# Autodesk Inventor assembly: liftMotorWithPotMounted
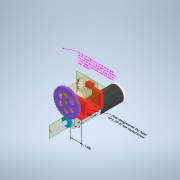
[picture p0: Inventor's stored thumbnail of the model, 180x180]
Saved by Autodesk Inventor 2020.2 (Build 242310000, 310)
## iProperties
Created: 2019-11-21
Part Number: liftMotorWithPotMounted
Document SubType Name: Assembly
Designer: steele
Author: steele
## Documents named in this file (9)
- C:\git\CAD-Development\robSteele\liftSpool\liftMotorWithPotMounted.iam
- C:\git\CAD-Development\robSteele\liftSpool\am-3762 - 36_1 - CIM Sport.iam
- C:\git\CAD-Development\robSteele\liftSpool\plateForPot.ipt
- C:\git\CAD-Development\robSteele\liftSpool\PotHolderAssembly.iam
- C:\git\CAD-Development\robSteele\liftSpool\liftMotorWithPotMounted\Design Accelerator\Spur Gears1.iam
- C:\git\CAD-Development\robSteele\liftSpool\spoolV09.ipt
- C:\git\CAD-Development\robSteele\liftSpool\am-0255+2.5inch+CIM+Motor.ipt
- C:\git\CAD-Development\robSteele\liftSpool\WormGearDriveForPot.iam
- C:\git\CAD-Development\robSteele\liftSpool\3_8_inchSteelShaft.ipt
## Components (8 placed, 8 different names)
1. am-3762 - 36_1 - CIM Sport:1 [sub-assembly] — Mate:1, Mate:2, Mate:3, Insert:1, Flush:1, Insert:2, Mate:4, Mate:5
2. plateForPot:1 — Mate:1, Mate:2, Mate:3
3. PotHolderAssembly:1 [sub-assembly] — Insert:5
4. Spur Gears:1 [sub-assembly] — Flush:1, Mate:4, Mate:5, Insert:3
5. spoolV09:1 — Insert:1
6. am-0255+2.5inch+CIM+Motor:1 — Insert:2
7. WormGearDriveForPot:1 [sub-assembly] — Insert:4, Insert:5
8. 3_8_inchSteelShaft:1 — Insert:3, Insert:4
## Relationships (11: Mate 5, Insert 5, Flush 1)
- Mate:1: am-3762 - 36_1 - CIM Sport:1 ↔ plateForPot:1
- Mate:2: am-3762 - 36_1 - CIM Sport:1 ↔ plateForPot:1
- Mate:3: am-3762 - 36_1 - CIM Sport:1 ↔ plateForPot:1
- Insert:1: am-3762 - 36_1 - CIM Sport:1 ↔ spoolV09:1
- Flush:1: am-3762 - 36_1 - CIM Sport:1 ↔ Spur Gears:1
- Insert:2: am-3762 - 36_1 - CIM Sport:1 ↔ am-0255+2.5inch+CIM+Motor:1
- Mate:4: am-3762 - 36_1 - CIM Sport:1 ↔ Spur Gears:1
- Mate:5: am-3762 - 36_1 - CIM Sport:1 ↔ Spur Gears:1
- Insert:3: Spur Gears:1 ↔ 3_8_inchSteelShaft:1
- Insert:4 (-9.906 mm): WormGearDriveForPot:1 ↔ 3_8_inchSteelShaft:1
- Insert:5: PotHolderAssembly:1 ↔ WormGearDriveForPot:1
